# Autodesk Inventor assembly: Clamp
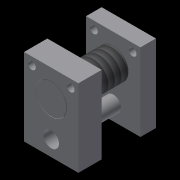
[picture p0: Inventor's stored thumbnail of the model, 180x180]
Saved by Autodesk Inventor 2017 (Build 210142000, 142)
## iProperties
Created: 2016-12-23
Part Number: Clamp
Document SubType Name: Assembly
Designer: David Kopala
Author: David Kopala
## Documents named in this file (4)
- \\Mac\Home\Documents\Drone\Drone\3D Models\Project\Chasis_02\Clamp\Clamp.iam
- \\Mac\Home\Documents\Drone\Drone\3D Models\Project\Chasis_02\Clamp\EndHole.ipt
- \\Mac\Home\Documents\Drone\Drone\3D Models\Project\Chasis_02\Clamp\Screw.ipt
- \\Mac\Home\Documents\Drone\Drone\3D Models\Project\Chasis_02\Clamp\Slider.ipt
## Components (3 placed, 3 different names)
1. EndHole:1 — Insert:1
2. Screw:1 — Insert:1, Insert:2
3. Slider:1 — Insert:2
## Relationships (2: Insert 2)
- Insert:1: EndHole:1 ↔ Screw:1
- Insert:2: Screw:1 ↔ Slider:1
